# Autodesk Inventor assembly: 000-belt_liner_v2
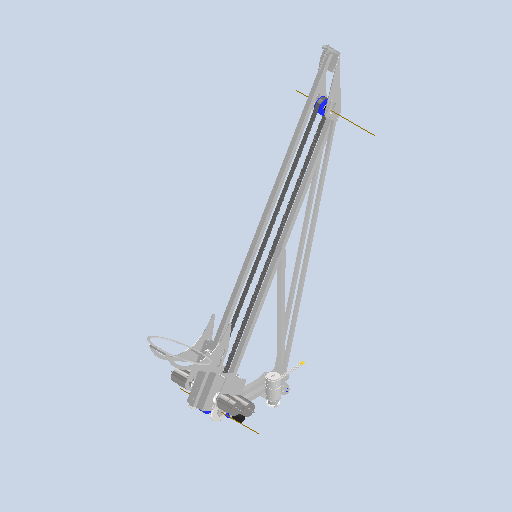
[picture p0: Inventor's stored thumbnail of the model, 512x512]
Saved by Autodesk Inventor 2025.2 (Build 292293000, 293)
## iProperties
Created: 2025-01-05
Part Number: 000-belt_liner_v2
Document SubType Name: Assembly
Designer: haruy
Mass: 5567.97 g
Surface Area: 9797.11 cm^2
Volume: 1342.66 cm^3
Density: 4.14697 g/cm^3
Author: haruy
## Documents named in this file (53)
- C:\Users\haruy\Documents\ロボコン\NHK2025\cad\nagahisa\belt_liner\000-belt_liner_v2.iam
- C:\Users\haruy\Documents\ロボコン\NHK2025\cad\nagahisa\belt_liner\belt_liner_v2_ASP_Base.ipt
- C:\Users\haruy\Documents\ロボコン\NHK2025\cad\nagahisa\belt_liner\belt_liner_v2_Plate_1.ipt
- C:\Users\haruy\Documents\ロボコン\NHK2025\cad\nagahisa\belt_liner\belt_liner_v2_Plate_2.ipt
- C:\Users\haruy\Documents\ロボコン\NHK2025\cad\nagahisa\belt_liner\belt_liner_v2_B_unit.ipt
- C:\Users\haruy\Documents\ロボコン\NHK2025\cad\nagahisa\belt_liner\belt_liner_v2_Plate_3.ipt
- C:\Users\haruy\Documents\ロボコン\NHK2025\cad\nagahisa\belt_liner\belt_liner_v2_Plate_4.ipt
- C:\Users\haruy\Documents\ロボコン\NHK2025\cad\nagahisa\belt_liner\belt_liner_v2_Plate_5.ipt
- C:\Users\haruy\Documents\ロボコン\NHK2025\cad\nagahisa\belt_liner\belt_liner_v2_Plate_6.ipt
- C:\Users\haruy\Documents\ロボコン\NHK2025\cad\nagahisa\belt_liner\belt_liner_v2_Plate_7.ipt
- C:\Users\haruy\Documents\ロボコン\NHK2025\cad\nagahisa\belt_liner\belt_liner_v2_Pom_r.ipt
- C:\Users\haruy\Documents\ロボコン\NHK2025\cad\nagahisa\belt_liner\belt_liner_v2_Plate_8.ipt
- C:\Users\haruy\Documents\ロボコン\NHK2025\cad\nagahisa\belt_liner\belt_liner_v2_Plate_9.ipt
- C:\Users\haruy\Documents\ロボコン\NHK2025\cad\nagahisa\belt_liner\belt_liner_v2_Plate_10.ipt
- C:\Users\haruy\Documents\ロボコン\NHK2025\cad\nagahisa\belt_liner\belt_liner_v2_Plate_11.ipt
- C:\Users\haruy\Documents\ロボコン\NHK2025\cad\nagahisa\belt_liner\belt_liner_v1_Plate_9.ipt
- C:\Users\haruy\Documents\ロボコン\NHK2025\cad\nagahisa\belt_liner\belt_liner_v2_Plate_12.ipt
- C:\Users\haruy\Documents\ロボコン\NHK2025\cad\nagahisa\belt_liner\C-SHFMQ20_b.ipt
- C:\Users\haruy\Documents\ロボコン\NHK2025\cad\nagahisa\belt_liner\roja-v1-3DP-rotate-spesa.ipt
- C:\Users\haruy\Documents\ロボコン\NHK2025\cad\nagahisa\belt_liner\roja-v1-Shaft-rotate.ipt
- C:\Users\haruy\Documents\ロボコン\NHK2025\cad\nagahisa\belt_liner\belt_liner_v2_Plate_13.ipt
- C:\Users\haruy\Documents\ロボコン\NHK2025\cad\nagahisa\belt_liner\belt_liner_v2_B_unit-2.ipt
- C:\Users\haruy\Documents\ロボコン\NHK2025\cad\nagahisa\belt_liner\belt_liner_v2_Plate_14.ipt
- C:\Users\haruy\Documents\ロボコン\NHK2025\cad\nagahisa\belt_liner\belt_liner_v2_Plate_15.ipt
- C:\Users\haruy\Documents\ロボコン\NHK2025\cad\000_parts\モーター\robomaster\M3508.ipt
- C:\Users\haruy\Documents\ロボコン\NHK2025\cad\nagahisa\belt_liner\000-belt_liner_v2\デザイン アクセラレータ\平歯車1.iam
- C:\Users\haruy\Documents\ロボコン\NHK2025\cad\nagahisa\belt_liner\belt_liner_v1_shaft_spesa-25.ipt
- C:\Users\haruy\Documents\ロボコン\NHK2025\cad\nagahisa\belt_liner\rs735.ipt
- C:\Users\haruy\Documents\ロボコン\NHK2025\cad\000_parts\エンコーダー\encoder v2.ipt
- C:\Users\haruy\Documents\ロボコン\NHK2025\cad\nagahisa\belt_liner\setcorer_5-10-22.ipt
- C:\Users\haruy\Documents\ロボコン\NHK2025\cad\nagahisa\belt_liner\000-belt_liner_v1\デザイン アクセラレータ\平歯車3.iam
- C:\Users\haruy\Documents\ロボコン\NHK2025\cad\nagahisa\belt_liner\belt_liner_v2_shaft_spesa-30.ipt
- C:\Users\haruy\Documents\ロボコン\NHK2025\cad\000_parts\ベアリング\10\bear_10_15_sn.ipt
- C:\Users\haruy\Documents\ロボコン\NHK2025\cad\nagahisa\belt_liner\SCBRJ10-13.iam
- C:\Users\haruy\Documents\ロボコン\NHK2025\cad\nagahisa\belt_liner\belt_liner_v2_shaft_1.ipt
- C:\Users\haruy\Documents\ロボコン\NHK2025\cad\nagahisa\belt_liner\SCSWJ10-6.iam
- C:\Users\haruy\Documents\ロボコン\NHK2025\cad\nagahisa\belt_liner\SSCSW10-10b.ipt
- C:\Users\haruy\Documents\ロボコン\NHK2025\cad\nagahisa\belt_liner\000-belt_liner_v2\デザイン アクセラレータ\平歯車2.iam
- C:\Users\haruy\Documents\ロボコン\NHK2025\cad\nagahisa\belt_liner\000-belt_liner_v2\デザイン アクセラレータ\平歯車3.iam
- C:\Users\haruy\Documents\ロボコン\NHK2025\cad\nagahisa\belt_liner\belt_liner_v2_Plate_18.ipt
- C:\Users\haruy\Documents\ロボコン\NHK2025\cad\nagahisa\belt_liner\belt_liner_v2_Plate_19.ipt
- C:\Users\haruy\Documents\ロボコン\NHK2025\cad\nagahisa\belt_liner\belt_liner_v2_Plate_20.ipt
- C:\Users\haruy\Documents\ロボコン\NHK2025\cad\nagahisa\belt_liner\000-belt_liner_v2\デザイン アクセラレータ\歯付きベルト伝達2.iam
- C:\Users\haruy\Documents\ロボコン\NHK2025\cad\nagahisa\belt_liner\belt_liner_v2_3DP_P-3-F.ipt
- C:\Users\haruy\Documents\ロボコン\NHK2025\cad\nagahisa\belt_liner\belt_liner_v2_3DP_P-4-F.ipt
- C:\Users\haruy\Documents\ロボコン\NHK2025\cad\nagahisa\belt_liner\belt_liner_v2_3DP_P-5-F.ipt
- C:\Users\haruy\Documents\ロボコン\NHK2025\cad\nagahisa\belt_liner\belt_liner_v2_3DP_P-6-F.ipt
- C:\Users\haruy\Documents\ロボコン\NHK2025\cad\nagahisa\belt_liner\belt_liner_v2_Plate_21.ipt
- C:\Users\haruy\Documents\ロボコン\NHK2025\cad\nagahisa\belt_liner\belt_liner_v2_shaft_2.ipt
- C:\Users\haruy\Documents\ロボコン\NHK2025\cad\nagahisa\belt_liner\000-belt_liner_v2\デザイン アクセラレータ\平歯車4.iam
- C:\Users\haruy\Documents\ロボコン\NHK2025\cad\nagahisa\belt_liner\belt_liner_v4_Plate_1.ipt
- C:\Users\haruy\Documents\ロボコン\NHK2025\cad\nagahisa\belt_liner\belt_liner-gear-v4-1.iam
- C:\Users\haruy\Documents\ロボコン\NHK2025\cad\nagahisa\belt_liner\belt_liner_v4_Plate_2.ipt
## Components (91 placed, 48 different names)
1. belt_liner_v2_ASP_Base:1 — 正接:1, 正接:2, 正接:3, 正接:4, 角度:1, 角度:2, 挿入:39, 挿入:40, 挿入:41, 挿入:42, 挿入:43, 挿入:44, 挿入:45, 挿入:46, 挿入:59, 挿入:60, 挿入:65, 挿入:66, 挿入:71, 挿入:72, フラッシュ:1, 挿入:124, 挿入:127, 挿入:128, 挿入:129, 挿入:130
2. belt_liner_v2_Plate_1:1 — 挿入:51, 挿入:52, 挿入:101, 挿入:102, 挿入:107, 挿入:170
3. belt_liner_v2_Plate_1:2 — 挿入:53, 挿入:54, 挿入:78, 挿入:79, 挿入:106
4. belt_liner_v2_Plate_2:1 — 挿入:47, 挿入:48, 挿入:55, 挿入:56
5. belt_liner_v2_Plate_2:2 — 挿入:49, 挿入:50, 挿入:57, 挿入:58
6. belt_liner_v2_B_unit:1 — 挿入:21, 挿入:22, 挿入:23, 挿入:24, 正接:1, 正接:2, 正接:3, 正接:4, 挿入:141, 挿入:142, 挿入:143, 挿入:144, 挿入:145, 挿入:146, 挿入:147, 挿入:148
7. belt_liner_v2_Plate_3:1 — 挿入:21, 挿入:22, 角度:1, 角度:2
8. belt_liner_v2_Plate_4:1 — 挿入:23, 挿入:24, 挿入:25, 挿入:26, 挿入:27, 挿入:28, 挿入:29, 挿入:30, 挿入:31, 挿入:32
9. belt_liner_v2_Plate_5:1 — 挿入:25, 挿入:26
10. belt_liner_v2_Plate_5:2 — 挿入:27, 挿入:28
11. belt_liner_v2_Plate_6:1 — 挿入:29, 挿入:30, 挿入:33, 挿入:36
12. belt_liner_v2_Plate_6:2 — 挿入:31, 挿入:32, 挿入:34, 角度:3, 挿入:35
13. belt_liner_v2_Plate_7:1 — 挿入:35, 挿入:36, 角度:4, 挿入:162
14. belt_liner_v2_Plate_7:2 — 挿入:33, 挿入:34, 角度:3, 角度:4, 挿入:163
15. belt_liner_v2_Pom_r:1 — 挿入:162, 挿入:163
16. belt_liner_v2_Plate_8:1 — 挿入:45, 挿入:46, 挿入:51, 挿入:52, 挿入:53, 挿入:54
17. belt_liner_v2_Plate_9:1 — 挿入:43, 挿入:44
18. belt_liner_v2_Plate_10:1 — 挿入:41, 挿入:42
19. belt_liner_v2_Plate_11:1 — 挿入:39, 挿入:40, 挿入:47, 挿入:48, 挿入:49, 挿入:50, 挿入:159, 挿入:160
20. belt_liner_v1_Plate_9:1 — 挿入:57, 挿入:58
21. belt_liner_v1_Plate_9:2 — 挿入:55, 挿入:56
22. belt_liner_v2_Plate_12:1 — 挿入:59, 挿入:60, 挿入:61, 挿入:62
23. C-SHFMQ20_b:1 — 挿入:61, 挿入:62, 挿入:63, 挿入:64
24. roja-v1-3DP-rotate-spesa:1 — 挿入:63
25. roja-v1-Shaft-rotate:1 — 挿入:64
26. belt_liner_v2_Plate_13:1 — 挿入:65, 挿入:66, 挿入:67
27. belt_liner_v2_B_unit-2:1 — 挿入:67, 挿入:69, 挿入:70, 挿入:149, 挿入:150, 挿入:151, 挿入:152
28. belt_liner_v2_Plate_14:1 — 挿入:69, 挿入:70
29. belt_liner_v2_Plate_15:1 — 挿入:71, 挿入:72, 挿入:73, 挿入:153
30. M3508:1 — 挿入:73, メイト:1, 挿入:113, 挿入:153
31. 平歯車:1 [sub-assembly] — メイト:1, メイト:2
32. belt_liner_v1_shaft_spesa-25:1 — 挿入:79, 挿入:173
33. belt_liner_v1_shaft_spesa-25:2 — 挿入:172
34. belt_liner_v1_shaft_spesa-25:3 — 挿入:78, 挿入:171
35. rs735:1 — 挿入:93, 挿入:174
36. rs735:2 — 挿入:92, 挿入:175
37. rs735:3 — 挿入:90, 挿入:168
38. rs735:4 — 挿入:91, 挿入:167
39. encoder v2:1 — メイト:9, 挿入:166
40. setcorer_5-10-22:1 — 挿入:91, 挿入:95
41. setcorer_5-10-22:2 — 挿入:93, 挿入:97
42. setcorer_5-10-22:3 — 挿入:92, 挿入:96
43. setcorer_5-10-22:4 — 挿入:90, 挿入:94
44. 平歯車:2 [sub-assembly] — 挿入:94
45. 平歯車:3 [sub-assembly] — 挿入:95
46. 平歯車:4 [sub-assembly] — 挿入:97
47. 平歯車:5 [sub-assembly] — 挿入:96
48. belt_liner_v2_shaft_spesa-30:1 — 挿入:101, 挿入:164
49. belt_liner_v2_shaft_spesa-30:2 — 挿入:102, 挿入:165
50. belt_liner_v2_shaft_spesa-30:3 — 挿入:170
51. bear_10_15_sn:1 — 挿入:107, 挿入:109
52. bear_10_15_sn:2 — 挿入:106, 挿入:108, 挿入:110
53. SCBRJ10-13:1 [sub-assembly] — 挿入:108
54. SCBRJ10-13:2 [sub-assembly] — 挿入:109
55. belt_liner_v2_shaft_1:1 — 挿入:110, 挿入:111, 挿入:112, メイト:3, メイト:5
56. SCSWJ10-6:1 [sub-assembly] — 挿入:112, メイト:4, 挿入:169
57. SCSWJ10-6:2 [sub-assembly] — 挿入:111, メイト:6, 挿入:176
58. SSCSW10-10b:1 — 挿入:113, メイト:2
59. SCSWJ10-6:3 [sub-assembly] — 挿入:140
60. 平歯車:7 [sub-assembly] — メイト:3, メイト:4, フラッシュ:2
61. 平歯車:8 [sub-assembly] — メイト:5, メイト:6
62. bear_10_15_sn:3 — 挿入:123, 挿入:154
63. bear_10_15_sn:4 — 挿入:122
64. SCBRJ10-13:3 [sub-assembly] — 挿入:123
65. SCBRJ10-13:4 [sub-assembly] — 挿入:122, 挿入:124
66. belt_liner_v2_Plate_18:1 — 挿入:125, 挿入:126
67. belt_liner_v2_Plate_19:1 — 挿入:125, 挿入:126, メイト:7, メイト:8
68. belt_liner_v2_Plate_20:1 — 挿入:127, 挿入:128
69. belt_liner_v2_Plate_20:2 — 挿入:129, 挿入:130
70. 歯付きベルト伝達:1 [sub-assembly] — メイト:7, メイト:8, 挿入:140, 挿入:155, 挿入:156, 挿入:157, 挿入:158
71. belt_liner_v2_3DP_P-3-F:1 — 挿入:154, 挿入:155, 挿入:156
72. belt_liner_v2_3DP_P-4-F:1 — 挿入:157, 挿入:158
73. belt_liner_v2_3DP_P-5-F:1 — 挿入:141
74. belt_liner_v2_3DP_P-5-F:2 — 挿入:142
75. belt_liner_v2_3DP_P-5-F:3 — 挿入:143
76. belt_liner_v2_3DP_P-5-F:4 — 挿入:144
77. belt_liner_v2_3DP_P-5-F:5 — 挿入:148
78. belt_liner_v2_3DP_P-5-F:6 — 挿入:146
79. belt_liner_v2_3DP_P-5-F:7 — 挿入:147
80. belt_liner_v2_3DP_P-5-F:8 — 挿入:145
81. belt_liner_v2_3DP_P-6-F:1 — 挿入:149
82. belt_liner_v2_3DP_P-6-F:2 — 挿入:150
83. belt_liner_v2_3DP_P-6-F:3 — 挿入:151
84. belt_liner_v2_3DP_P-6-F:4 — 挿入:152
85. belt_liner_v2_Plate_21:1 — 挿入:159, 挿入:160, 挿入:161
86. belt_liner_v2_shaft_2:1 — 挿入:161
87. 平歯車:9 [sub-assembly] — メイト:9, フラッシュ:2
88. belt_liner_v4_Plate_1:1 — 挿入:164, 挿入:165, 挿入:166, 挿入:167, 挿入:168
89. belt_liner-gear-v4-1:1 [sub-assembly] — 挿入:169
90. belt_liner_v4_Plate_2:1 — 挿入:171, 挿入:172, 挿入:173, 挿入:174, 挿入:175
91. belt_liner-gear-v4-1:2 [sub-assembly] — 挿入:176
## Relationships (135: Insert 116, Mate 9, Tangent 4, Angle 4, Flush 2)
- 挿入:21 [Insert]: belt_liner_v2_B_unit:1 ↔ belt_liner_v2_Plate_3:1
- 挿入:22 [Insert]: belt_liner_v2_B_unit:1 ↔ belt_liner_v2_Plate_3:1
- 挿入:23 [Insert]: belt_liner_v2_B_unit:1 ↔ belt_liner_v2_Plate_4:1
- 挿入:24 [Insert]: belt_liner_v2_B_unit:1 ↔ belt_liner_v2_Plate_4:1
- 正接:1 [Tangent]: belt_liner_v2_ASP_Base:1 ↔ belt_liner_v2_B_unit:1
- 正接:2 [Tangent]: belt_liner_v2_ASP_Base:1 ↔ belt_liner_v2_B_unit:1
- 正接:3 [Tangent]: belt_liner_v2_ASP_Base:1 ↔ belt_liner_v2_B_unit:1
- 正接:4 [Tangent]: belt_liner_v2_ASP_Base:1 ↔ belt_liner_v2_B_unit:1
- 角度:1 [Angle] (0 deg): belt_liner_v2_ASP_Base:1 ↔ belt_liner_v2_Plate_3:1
- 角度:2 [Angle] (0 deg): belt_liner_v2_ASP_Base:1 ↔ belt_liner_v2_Plate_3:1
- 挿入:25 [Insert]: belt_liner_v2_Plate_4:1 ↔ belt_liner_v2_Plate_5:1
- 挿入:26 [Insert]: belt_liner_v2_Plate_4:1 ↔ belt_liner_v2_Plate_5:1
- 挿入:27 [Insert]: belt_liner_v2_Plate_4:1 ↔ belt_liner_v2_Plate_5:2
- 挿入:28 [Insert]: belt_liner_v2_Plate_4:1 ↔ belt_liner_v2_Plate_5:2
- 挿入:29 [Insert]: belt_liner_v2_Plate_4:1 ↔ belt_liner_v2_Plate_6:1
- 挿入:30 [Insert]: belt_liner_v2_Plate_4:1 ↔ belt_liner_v2_Plate_6:1
- 挿入:31 [Insert]: belt_liner_v2_Plate_4:1 ↔ belt_liner_v2_Plate_6:2
- 挿入:32 [Insert]: belt_liner_v2_Plate_4:1 ↔ belt_liner_v2_Plate_6:2
- 挿入:33 [Insert]: belt_liner_v2_Plate_6:1 ↔ belt_liner_v2_Plate_7:2
- 挿入:34 [Insert]: belt_liner_v2_Plate_6:2 ↔ belt_liner_v2_Plate_7:2
- 角度:3 [Angle] (0 deg): belt_liner_v2_Plate_6:2 ↔ belt_liner_v2_Plate_7:2
- 挿入:35 [Insert]: belt_liner_v2_Plate_6:2 ↔ belt_liner_v2_Plate_7:1
- 挿入:36 [Insert]: belt_liner_v2_Plate_6:1 ↔ belt_liner_v2_Plate_7:1
- 角度:4 [Angle] (0 deg): belt_liner_v2_Plate_7:1 ↔ belt_liner_v2_Plate_7:2
- 挿入:39 [Insert]: belt_liner_v2_ASP_Base:1 ↔ belt_liner_v2_Plate_11:1
- 挿入:40 [Insert]: belt_liner_v2_ASP_Base:1 ↔ belt_liner_v2_Plate_11:1
- 挿入:41 [Insert]: belt_liner_v2_ASP_Base:1 ↔ belt_liner_v2_Plate_10:1
- 挿入:42 [Insert]: belt_liner_v2_ASP_Base:1 ↔ belt_liner_v2_Plate_10:1
- 挿入:43 [Insert]: belt_liner_v2_ASP_Base:1 ↔ belt_liner_v2_Plate_9:1
- 挿入:44 [Insert]: belt_liner_v2_ASP_Base:1 ↔ belt_liner_v2_Plate_9:1
- 挿入:45 [Insert]: belt_liner_v2_ASP_Base:1 ↔ belt_liner_v2_Plate_8:1
- 挿入:46 [Insert]: belt_liner_v2_ASP_Base:1 ↔ belt_liner_v2_Plate_8:1
- 挿入:47 [Insert]: belt_liner_v2_Plate_2:1 ↔ belt_liner_v2_Plate_11:1
- 挿入:48 [Insert]: belt_liner_v2_Plate_2:1 ↔ belt_liner_v2_Plate_11:1
- 挿入:49 [Insert]: belt_liner_v2_Plate_2:2 ↔ belt_liner_v2_Plate_11:1
- 挿入:50 [Insert]: belt_liner_v2_Plate_2:2 ↔ belt_liner_v2_Plate_11:1
- 挿入:51 [Insert]: belt_liner_v2_Plate_1:1 ↔ belt_liner_v2_Plate_8:1
- 挿入:52 [Insert]: belt_liner_v2_Plate_1:1 ↔ belt_liner_v2_Plate_8:1
- 挿入:53 [Insert]: belt_liner_v2_Plate_1:2 ↔ belt_liner_v2_Plate_8:1
- 挿入:54 [Insert]: belt_liner_v2_Plate_1:2 ↔ belt_liner_v2_Plate_8:1
- 挿入:55 [Insert]: belt_liner_v2_Plate_2:1 ↔ belt_liner_v1_Plate_9:2
- 挿入:56 [Insert]: belt_liner_v2_Plate_2:1 ↔ belt_liner_v1_Plate_9:2
- 挿入:57 [Insert]: belt_liner_v2_Plate_2:2 ↔ belt_liner_v1_Plate_9:1
- 挿入:58 [Insert]: belt_liner_v2_Plate_2:2 ↔ belt_liner_v1_Plate_9:1
- 挿入:59 [Insert]: belt_liner_v2_ASP_Base:1 ↔ belt_liner_v2_Plate_12:1
- 挿入:60 [Insert]: belt_liner_v2_ASP_Base:1 ↔ belt_liner_v2_Plate_12:1
- 挿入:61 [Insert]: belt_liner_v2_Plate_12:1 ↔ C-SHFMQ20_b:1
- 挿入:62 [Insert]: belt_liner_v2_Plate_12:1 ↔ C-SHFMQ20_b:1
- 挿入:63 [Insert]: C-SHFMQ20_b:1 ↔ roja-v1-3DP-rotate-spesa:1
- 挿入:64 [Insert]: C-SHFMQ20_b:1 ↔ roja-v1-Shaft-rotate:1
- 挿入:65 [Insert]: belt_liner_v2_ASP_Base:1 ↔ belt_liner_v2_Plate_13:1
- 挿入:66 [Insert]: belt_liner_v2_ASP_Base:1 ↔ belt_liner_v2_Plate_13:1
- 挿入:67 [Insert]: belt_liner_v2_Plate_13:1 ↔ belt_liner_v2_B_unit-2:1
- 挿入:69 [Insert]: belt_liner_v2_B_unit-2:1 ↔ belt_liner_v2_Plate_14:1
- 挿入:70 [Insert]: belt_liner_v2_B_unit-2:1 ↔ belt_liner_v2_Plate_14:1
- 挿入:71 [Insert]: belt_liner_v2_ASP_Base:1 ↔ belt_liner_v2_Plate_15:1
- 挿入:72 [Insert]: belt_liner_v2_ASP_Base:1 ↔ belt_liner_v2_Plate_15:1
- 挿入:73 [Insert]: belt_liner_v2_Plate_15:1 ↔ M3508:1
- メイト:1 [Mate]: M3508:1 ↔ 平歯車:1
- 挿入:78 [Insert]: belt_liner_v2_Plate_1:2 ↔ belt_liner_v1_shaft_spesa-25:3
- 挿入:79 [Insert]: belt_liner_v2_Plate_1:2 ↔ belt_liner_v1_shaft_spesa-25:1
- 挿入:90 [Insert]: rs735:3 ↔ setcorer_5-10-22:4
- 挿入:91 [Insert]: rs735:4 ↔ setcorer_5-10-22:1
- 挿入:92 [Insert]: rs735:2 ↔ setcorer_5-10-22:3
- 挿入:93 [Insert]: rs735:1 ↔ setcorer_5-10-22:2
- 挿入:94 [Insert]: setcorer_5-10-22:4 ↔ 平歯車:2
- 挿入:95 [Insert]: setcorer_5-10-22:1 ↔ 平歯車:3
- 挿入:96 [Insert]: setcorer_5-10-22:3 ↔ 平歯車:5
- 挿入:97 [Insert]: setcorer_5-10-22:2 ↔ 平歯車:4
- 挿入:101 [Insert]: belt_liner_v2_Plate_1:1 ↔ belt_liner_v2_shaft_spesa-30:1
- 挿入:102 [Insert]: belt_liner_v2_Plate_1:1 ↔ belt_liner_v2_shaft_spesa-30:2
- 挿入:106 [Insert]: belt_liner_v2_Plate_1:2 ↔ bear_10_15_sn:2
- 挿入:107 [Insert]: belt_liner_v2_Plate_1:1 ↔ bear_10_15_sn:1
- 挿入:108 [Insert]: bear_10_15_sn:2 ↔ SCBRJ10-13:1
- 挿入:109 [Insert]: bear_10_15_sn:1 ↔ SCBRJ10-13:2
- 挿入:110 [Insert] (-19 mm): bear_10_15_sn:2 ↔ belt_liner_v2_shaft_1:1
- 挿入:111 [Insert]: belt_liner_v2_shaft_1:1 ↔ SCSWJ10-6:2
- 挿入:112 [Insert]: belt_liner_v2_shaft_1:1 ↔ SCSWJ10-6:1
- 挿入:113 [Insert] (5 mm): M3508:1 ↔ SSCSW10-10b:1
- メイト:2 [Mate]: 平歯車:1 ↔ SSCSW10-10b:1
- メイト:3 [Mate]: belt_liner_v2_shaft_1:1 ↔ 平歯車:7
- メイト:4 [Mate]: SCSWJ10-6:1 ↔ 平歯車:7
- フラッシュ:1 [Flush] (-7.5 mm): belt_liner_v2_ASP_Base:1
- メイト:5 [Mate]: belt_liner_v2_shaft_1:1 ↔ 平歯車:8
- メイト:6 [Mate]: SCSWJ10-6:2 ↔ 平歯車:8
- 挿入:122 [Insert]: bear_10_15_sn:4 ↔ SCBRJ10-13:4
- 挿入:123 [Insert]: bear_10_15_sn:3 ↔ SCBRJ10-13:3
- 挿入:124 [Insert] (-14.5 mm): belt_liner_v2_ASP_Base:1 ↔ SCBRJ10-13:4
- 挿入:125 [Insert]: belt_liner_v2_Plate_18:1 ↔ belt_liner_v2_Plate_19:1
- 挿入:126 [Insert]: belt_liner_v2_Plate_18:1 ↔ belt_liner_v2_Plate_19:1
- 挿入:127 [Insert]: belt_liner_v2_ASP_Base:1 ↔ belt_liner_v2_Plate_20:1
- 挿入:128 [Insert]: belt_liner_v2_ASP_Base:1 ↔ belt_liner_v2_Plate_20:1
- 挿入:129 [Insert]: belt_liner_v2_ASP_Base:1 ↔ belt_liner_v2_Plate_20:2
- 挿入:130 [Insert]: belt_liner_v2_ASP_Base:1 ↔ belt_liner_v2_Plate_20:2
- メイト:7 [Mate]: belt_liner_v2_Plate_19:1 ↔ 歯付きベルト伝達:1
- メイト:8 [Mate]: belt_liner_v2_Plate_19:1 ↔ 歯付きベルト伝達:1
- 挿入:140 [Insert]: SCSWJ10-6:3 ↔ 歯付きベルト伝達:1
- 挿入:141 [Insert]: belt_liner_v2_B_unit:1 ↔ belt_liner_v2_3DP_P-5-F:1
- 挿入:142 [Insert]: belt_liner_v2_B_unit:1 ↔ belt_liner_v2_3DP_P-5-F:2
- 挿入:143 [Insert]: belt_liner_v2_B_unit:1 ↔ belt_liner_v2_3DP_P-5-F:3
- 挿入:144 [Insert]: belt_liner_v2_B_unit:1 ↔ belt_liner_v2_3DP_P-5-F:4
- 挿入:145 [Insert]: belt_liner_v2_B_unit:1 ↔ belt_liner_v2_3DP_P-5-F:8
- 挿入:146 [Insert]: belt_liner_v2_B_unit:1 ↔ belt_liner_v2_3DP_P-5-F:6
- 挿入:147 [Insert]: belt_liner_v2_B_unit:1 ↔ belt_liner_v2_3DP_P-5-F:7
- 挿入:148 [Insert]: belt_liner_v2_B_unit:1 ↔ belt_liner_v2_3DP_P-5-F:5
- 挿入:149 [Insert]: belt_liner_v2_B_unit-2:1 ↔ belt_liner_v2_3DP_P-6-F:1
- 挿入:150 [Insert]: belt_liner_v2_B_unit-2:1 ↔ belt_liner_v2_3DP_P-6-F:2
- 挿入:151 [Insert]: belt_liner_v2_B_unit-2:1 ↔ belt_liner_v2_3DP_P-6-F:3
- 挿入:152 [Insert]: belt_liner_v2_B_unit-2:1 ↔ belt_liner_v2_3DP_P-6-F:4
- 挿入:153 [Insert]: belt_liner_v2_Plate_15:1 ↔ M3508:1
- 挿入:154 [Insert]: bear_10_15_sn:3 ↔ belt_liner_v2_3DP_P-3-F:1
- 挿入:155 [Insert]: 歯付きベルト伝達:1 ↔ belt_liner_v2_3DP_P-3-F:1
- 挿入:156 [Insert]: 歯付きベルト伝達:1 ↔ belt_liner_v2_3DP_P-3-F:1
- 挿入:157 [Insert]: 歯付きベルト伝達:1 ↔ belt_liner_v2_3DP_P-4-F:1
- 挿入:158 [Insert]: 歯付きベルト伝達:1 ↔ belt_liner_v2_3DP_P-4-F:1
- 挿入:159 [Insert]: belt_liner_v2_Plate_11:1 ↔ belt_liner_v2_Plate_21:1
- 挿入:160 [Insert]: belt_liner_v2_Plate_11:1 ↔ belt_liner_v2_Plate_21:1
- 挿入:161 [Insert] (-10 mm): belt_liner_v2_Plate_21:1 ↔ belt_liner_v2_shaft_2:1
- メイト:9 [Mate]: encoder v2:1 ↔ 平歯車:9
- フラッシュ:2 [Flush]: 平歯車:7 ↔ 平歯車:9
- 挿入:162 [Insert]: belt_liner_v2_Plate_7:1 ↔ belt_liner_v2_Pom_r:1
- 挿入:163 [Insert]: belt_liner_v2_Plate_7:2 ↔ belt_liner_v2_Pom_r:1
- 挿入:164 [Insert]: belt_liner_v2_shaft_spesa-30:1 ↔ belt_liner_v4_Plate_1:1
- 挿入:165 [Insert]: belt_liner_v2_shaft_spesa-30:2 ↔ belt_liner_v4_Plate_1:1
- 挿入:166 [Insert]: encoder v2:1 ↔ belt_liner_v4_Plate_1:1
- 挿入:167 [Insert]: rs735:4 ↔ belt_liner_v4_Plate_1:1
- 挿入:168 [Insert]: rs735:3 ↔ belt_liner_v4_Plate_1:1
- 挿入:169 [Insert]: SCSWJ10-6:1 ↔ belt_liner-gear-v4-1:1
- 挿入:170 [Insert]: belt_liner_v2_Plate_1:1 ↔ belt_liner_v2_shaft_spesa-30:3
- 挿入:171 [Insert]: belt_liner_v1_shaft_spesa-25:3 ↔ belt_liner_v4_Plate_2:1
- 挿入:172 [Insert]: belt_liner_v1_shaft_spesa-25:2 ↔ belt_liner_v4_Plate_2:1
- 挿入:173 [Insert]: belt_liner_v1_shaft_spesa-25:1 ↔ belt_liner_v4_Plate_2:1
- 挿入:174 [Insert]: rs735:1 ↔ belt_liner_v4_Plate_2:1
- 挿入:175 [Insert]: rs735:2 ↔ belt_liner_v4_Plate_2:1
- 挿入:176 [Insert]: SCSWJ10-6:2 ↔ belt_liner-gear-v4-1:2
